# Autodesk Inventor assembly: mobile_robot_car
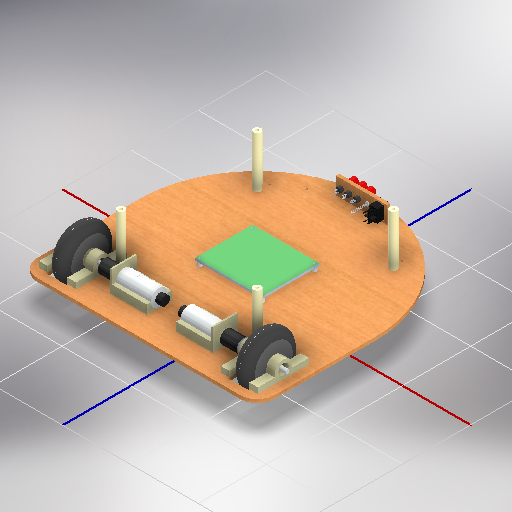
[picture p0: Inventor's stored thumbnail of the model, 512x512]
Saved by Autodesk Inventor 2026 (Build 300175050, 175E)
## iProperties
Created: 2025-06-05
Part Number: mobile_robot_car
Document SubType Name: Assembly
Designer: satom
Author: satom
## Documents named in this file (47)
- C:\Users\satom\Desktop\Robot\CAD\Inventor\mobile_robot_car.iam
- C:\Users\satom\Desktop\Robot\CAD\Inventor\C - Chassis\layer1_new.ipt
- C:\Users\satom\Desktop\Robot\CAD\Inventor\D - DriveTrain\motor_holder.ipt
- C:\Users\satom\Desktop\Robot\CAD\Inventor\D - DriveTrain\wheel_bearing.ipt
- C:\Users\satom\Desktop\Robot\CAD\Inventor\D - DriveTrain\wheel_mount.ipt
- C:\Users\satom\Desktop\Robot\CAD\Inventor\C - Chassis\3inch_standoff.ipt
- C:\Users\satom\Desktop\Robot\CAD\Inventor\solidworks\D - DriveTrain\motor\motor\motor.ipt
- C:\Users\satom\Desktop\Robot\CAD\Inventor\solidworks\D - DriveTrain\shaft_coupler\shaft_coupler\shaft_coupler.ipt
- C:\Users\satom\Desktop\Robot\CAD\Inventor\solidworks\D - DriveTrain\drive_shaft\drive_shaft\drive_shaft.ipt
- C:\Users\satom\Desktop\Robot\CAD\Inventor\solidworks\D - DriveTrain\ball_bearing\ball_bearing\ball_bearing.ipt
- C:\Users\satom\Desktop\Robot\CAD\Inventor\solidworks\E - Electronics\Main Board\Main Board\Main Board.ipt
- C:\Users\satom\Desktop\Robot\CAD\Inventor\solidworks\E - Electronics\NiMH_battery\NiMH_battery\NiMH_battery.ipt
- C:\Users\satom\Desktop\Robot\CAD\Inventor\C - Chassis\layer2_new.ipt
- C:\Users\satom\Desktop\Robot\CAD\Inventor\solidworks\E - Electronics\IMU breakout\IMU breakout\IMU breakout.ipt
- C:\Users\satom\Desktop\Robot\CAD\Inventor\C - Chassis\layer3_new.ipt
- C:\Users\satom\Desktop\Robot\CAD\Inventor\C - Chassis\9inch_spacer.ipt
- C:\Users\satom\Desktop\Robot\CAD\Inventor\C - Chassis\layer4_new.ipt
- C:\Users\satom\Desktop\Robot\CAD\Inventor\C - Chassis\layer5_new.ipt
- C:\Users\satom\Desktop\Robot\CAD\Inventor\C - Chassis\layer6_new.ipt
- C:\Users\satom\Desktop\Robot\CAD\Inventor\C - Chassis\3.5inch_standoff.ipt
- C:\Users\satom\Desktop\Robot\CAD\Inventor\solidworks\Display\Arducam_assembly\Arducam_assembly\Arducam_assembly.ipt
- C:\Users\satom\Desktop\Robot\CAD\Inventor\C - Chassis\LiDAR_plate.ipt
- C:\Users\satom\Desktop\Robot\CAD\Inventor\solidworks\E - Electronics\A2_LIDAR\A2_LIDAR\A2_LIDAR.ipt
- C:\Users\satom\Desktop\Robot\CAD\Inventor\C - Chassis\control_panel.ipt
- C:\Users\satom\Desktop\Robot\CAD\Inventor\E - Electronics\status_LED\status_LED\status_LED.ipt
- C:\Users\satom\Desktop\Robot\CAD\Inventor\E - Electronics\rocker_switch\rocker_switch\rocker_switch.ipt
- C:\Users\satom\Desktop\Robot\CAD\Inventor\E - Electronics\button\button\button.ipt
- C:\Users\satom\Desktop\Robot\CAD\Inventor\E - Electronics\microphone_casing.ipt
- C:\Users\satom\Desktop\Robot\CAD\Inventor\E - Electronics\microphone_casing_back.ipt
- C:\Users\satom\Desktop\Robot\CAD\Inventor\C - Chassis\display_top_support_left.ipt
- C:\Users\satom\Desktop\Robot\CAD\Inventor\C - Chassis\display_top_support_right.ipt
- C:\Users\satom\Desktop\Robot\CAD\Inventor\solidworks\Display\monitor\monitor\monitor.ipt
- C:\Users\satom\Desktop\Robot\CAD\Inventor\C - Chassis\display_bottom_support_left.ipt
- C:\Users\satom\Desktop\Robot\CAD\Inventor\C - Chassis\display_bottom_support_right.ipt
- C:\Users\satom\Desktop\Robot\CAD\Inventor\E - Electronics\NiMH_Holder_Front.ipt
- C:\Users\satom\Desktop\Robot\CAD\Inventor\E - Electronics\NiMH_Holder_Back.ipt
- C:\Users\satom\Desktop\Robot\CAD\Inventor\E - Electronics\jetson_orin_nano_holder_corner_1.ipt
- C:\Users\satom\Desktop\Robot\CAD\Inventor\E - Electronics\jetson_orin_nano_holder_corner_2.ipt
- C:\Users\satom\Desktop\Robot\CAD\Inventor\E - Electronics\orin_nano\orin_nano\orin_nano.ipt
- C:\Users\satom\Desktop\Robot\CAD\Inventor\E - Electronics\1-4_inch_standoff.ipt
- C:\Users\satom\Desktop\Robot\CAD\Inventor\E - Electronics\astra_holder.ipt
- C:\Users\satom\Desktop\Robot\CAD\Inventor\D - DriveTrain\wheel_80mm.ipt
- C:\Users\satom\Desktop\Robot\CAD\Inventor\D - DriveTrain\wheel_spacer_2.5mm.ipt
- C:\Users\satom\Desktop\Robot\CAD\Inventor\C - Chassis\foam_bumper_circular.ipt
- C:\Users\satom\Desktop\Robot\CAD\Inventor\C - Chassis\foam_bumper_bottom.ipt
- C:\Users\satom\Desktop\Robot\CAD\Inventor\solidworks\E - Electronics\Lion_5V\Lion_5V\Lion_5V.ipt
- C:\Users\satom\Desktop\Robot\CAD\Inventor\C - Chassis\ball_caster.ipt
## Components (103 placed, 46 different names)
1. layer1_new:1 — Mate:1, Mate:2, Mate:3, Mate:4, Mate:5, Mate:6, Mate:8, Mate:9, Mate:10, Mate:11, Mate:12, Mate:13, Mate:14, Mate:15, Mate:18, Mate:19, Mate:20, Mate:21, Mate:22, Mate:23, Mate:24, Mate:25, Mate:33, Mate:34, Mate:210, Mate:211, Mate:212, Mate:297, Mate:298, Mate:299, Mate:300, Mate:301, Mate:302, Mate:303, Mate:304, Mate:348, Mate:349, Mate:350, Mate:351, Mate:352, Mate:353
2. motor_holder:1 — Mate:1, Mate:29, Mate:30, Mate:34
3. motor_holder:2 — Mate:2, Mate:31, Mate:32, Mate:33
4. wheel_bearing:1 — Mate:5, Mate:12, Mate:13, Mate:43, Mate:44
5. wheel_bearing:2 — Mate:6, Mate:10, Mate:11, Mate:50, Mate:51
6. wheel_bearing:3 — Mate:4, Mate:14, Mate:15, Mate:45, Mate:46
7. wheel_bearing:4 — Mate:3, Mate:8, Mate:9, Mate:48, Mate:49
8. wheel_mount:1 — Mate:62, Mate:321, Mate:323
9. wheel_mount:2 — Mate:64, Mate:322, Mate:324
10. wheel_mount:3 — Mate:325, Mate:326
11. wheel_mount:4 — Mate:61, Mate:63, Mate:327, Mate:328
12. 3inch_standoff:1 — Mate:18, Mate:24, Mate:82
13. 3inch_standoff:2 — Mate:19, Mate:25, Mate:79, Mate:81
14. 3inch_standoff:3 — Mate:21, Mate:23, Mate:83
15. 3inch_standoff:4 — Mate:20, Mate:22, Mate:80
16. motor:1 — Mate:29, Mate:30, Mate:35, Mate:37
17. motor:2 — Mate:31, Mate:32, Mate:36, Mate:38
18. shaft_coupler:1 — Mate:36, Mate:38, Mate:39, Mate:41
19. shaft_coupler:2 — Mate:35, Mate:37, Mate:40, Mate:42
20. drive_shaft:1 — Mate:39, Mate:41, Mate:62, Mate:329, Mate:330
21. drive_shaft:2 — Mate:40, Mate:42, Mate:61, Mate:333, Mate:334
22. ball_bearing:1 — Mate:50, Mate:51, Mate:331
23. ball_bearing:2 — Mate:45, Mate:46, Mate:335
24. ball_bearing:3 — Mate:43, Mate:44, Mate:63, Mate:336
25. ball_bearing:4 — Mate:48, Mate:49, Mate:64, Mate:332
26. Main Board:1 — Mate:305, Mate:306, Mate:307
27. NiMH_battery:1 — Mate:265, Mate:266
28. NiMH_battery:2 — Mate:273, Mate:274
29. layer2_new:1 — Mate:79, Mate:80, Mate:81, Mate:82, Mate:83, Mate:95, Mate:96, Mate:97, Mate:98, Mate:99, Mate:100, Mate:101, Mate:102, Mate:259, Mate:260, Mate:261, Mate:262, Mate:263, Mate:264, Mate:267, Mate:268, Mate:269, Mate:270, Mate:271, Mate:272, Mate:275, Mate:276, Mate:277, Mate:282, Mate:283, Mate:284, Mate:285, Mate:286, Mate:287, Mate:288, Mate:289, Mate:290, Mate:308, Mate:309, Mate:310, Mate:311, Mate:312, Mate:313, Mate:345, Mate:346, Mate:347, Mate:354
30. IMU breakout:1 — Mate:314, Mate:315, Mate:316, Mate:317
31. 3inch_standoff:5 — Mate:97, Mate:101, Mate:103, Mate:104
32. 3inch_standoff:6 — Mate:96, Mate:102
33. 3inch_standoff:7 — Mate:98, Mate:99
34. 3inch_standoff:8 — Mate:95, Mate:100, Mate:105
35. layer3_new:1 — Mate:103, Mate:104, Mate:105, Mate:106, Mate:107, Mate:108, Mate:109, Mate:110, Mate:111, Mate:112, Mate:113, Mate:114, Mate:115, Mate:116, Mate:117, Mate:118, Mate:119, Mate:120, Mate:121, Mate:337, Mate:338
36. 9inch_spacer:1 — Mate:106, Mate:116, Mate:117, Mate:118, Mate:126, Mate:127
37. 9inch_spacer:2 — Mate:107, Mate:119, Mate:120, Mate:121, Mate:122, Mate:123, Mate:124, Mate:125
38. 9inch_spacer:3 — Mate:108, Mate:110, Mate:111, Mate:112, Mate:130, Mate:131
39. 9inch_spacer:4 — Mate:109, Mate:113, Mate:114, Mate:115, Mate:128, Mate:129
40. layer4_new:1 — Mate:122, Mate:123, Mate:124, Mate:125, Mate:126, Mate:127, Mate:128, Mate:129, Mate:130, Mate:131, Mate:132, Mate:133, Mate:134, Mate:135, Mate:136, Mate:137, Mate:138, Mate:139, Mate:140, Mate:141, Mate:142, Mate:143, Mate:144, Mate:145, Mate:146, Mate:147, Mate:339, Mate:340
41. 9inch_spacer:5 — Mate:135, Mate:145, Mate:146, Mate:147, Mate:148, Mate:152, Mate:153, Mate:154
42. 9inch_spacer:6 — Mate:134, Mate:142, Mate:143, Mate:144, Mate:155, Mate:156, Mate:157
43. 9inch_spacer:7 — Mate:133, Mate:136, Mate:137, Mate:138, Mate:158, Mate:159, Mate:160
44. 9inch_spacer:8 — Mate:132, Mate:139, Mate:140, Mate:141, Mate:149, Mate:150, Mate:151
45. layer5_new:1 — Mate:148, Mate:149, Mate:150, Mate:151, Mate:152, Mate:153, Mate:154, Mate:155, Mate:156, Mate:157, Mate:158, Mate:159, Mate:160, Mate:161, Mate:162, Mate:163, Mate:164, Mate:165, Mate:166, Mate:167, Mate:168, Mate:169, Mate:170, Mate:171, Mate:172, Mate:173, Mate:174, Mate:175, Mate:176, Mate:341, Mate:342
46. 9inch_spacer:9 — Mate:161, Mate:171, Mate:172, Mate:173, Mate:177, Mate:178, Mate:179, Mate:180, Mate:232
47. 9inch_spacer:10 — Mate:162, Mate:174, Mate:175, Mate:176, Mate:181, Mate:182, Mate:183, Mate:231
48. 9inch_spacer:11 — Mate:163, Mate:168, Mate:169, Mate:170, Mate:187, Mate:188, Mate:189
49. 9inch_spacer:12 — Mate:164, Mate:165, Mate:166, Mate:167, Mate:184, Mate:185, Mate:186
50. layer6_new:1 — Mate:177, Mate:178, Mate:179, Mate:180, Mate:181, Mate:182, Mate:183, Mate:184, Mate:185, Mate:186, Mate:187, Mate:188, Mate:189, Mate:190, Mate:191, Mate:192, Mate:193, Mate:194, Mate:195, Mate:196, Mate:197, Mate:198, Mate:199, Mate:233, Mate:234, Mate:235, Mate:236, Mate:239, Mate:243, Mate:318, Mate:319, Mate:320, Mate:343, Mate:344
51. 3.5inch_standoff:1 — Mate:191, Mate:194, Mate:201
52. 3.5inch_standoff:2 — Mate:190, Mate:197, Mate:203
53. 3.5inch_standoff:3 — Mate:192, Mate:196, Mate:200, Mate:204
54. 3.5inch_standoff:4 — Mate:193, Mate:195, Mate:202
55. Arducam_assembly:1 — Mate:198, Mate:199
56. LiDAR_plate:1 — Mate:200, Mate:201, Mate:202, Mate:203, Mate:204, Mate:205, Mate:206, Mate:207, Mate:208, Mate:209
57. A2_LIDAR:1 — Mate:205, Mate:206, Mate:207, Mate:208, Mate:209
58. control_panel:1 — Mate:210, Mate:211, Mate:212, Mate:213, Mate:214, Mate:215, Mate:216, Mate:217, Mate:218, Mate:219, Mate:220, Mate:221, Mate:222, Mate:223
59. status_LED:1 — Mate:213, Mate:214
60. rocker_switch:1 — Mate:215, Mate:216, Mate:217
61. button:1 — Mate:218, Mate:219
62. button:2 — Mate:221, Mate:222
63. button:3 — Mate:220, Mate:223
64. microphone_casing:1 — Mate:225, Mate:226, Mate:227
65. microphone_casing_back:1 — Mate:225, Mate:226, Mate:227, Mate:231
66. microphone_casing:2 — Mate:228, Mate:229, Mate:230
67. microphone_casing_back:2 — Mate:228, Mate:229, Mate:230, Mate:232
68. display_top_support_left:1 — Mate:233, Mate:234, Mate:238
69. display_top_support_right:1 — Mate:235, Mate:236, Mate:237, Mate:241
70. monitor:1 — Mate:237, Mate:238, Mate:241, Mate:242, Mate:244
71. display_bottom_support_left:1 — Mate:239, Mate:242
72. display_bottom_support_right:1 — Mate:243, Mate:244
73. NiMH_Holder_Front:1 — Mate:260, Mate:263, Mate:264, Mate:265
74. NiMH_Holder_Back:1 — Mate:259, Mate:261, Mate:262, Mate:266
75. NiMH_Holder_Back:2 — Mate:267, Mate:271, Mate:272, Mate:274
76. NiMH_Holder_Front:2 — Mate:268, Mate:269, Mate:270, Mate:273
77. jetson_orin_nano_holder_corner_1:1 — Mate:276, Mate:277, Mate:283
78. jetson_orin_nano_holder_corner_1:2 — Mate:275, Mate:282, Mate:284, Mate:292
79. jetson_orin_nano_holder_corner_2:1 — Mate:286, Mate:287, Mate:288
80. jetson_orin_nano_holder_corner_2:2 — Mate:285, Mate:289, Mate:290, Mate:291, Mate:293
81. orin_nano:1 — Mate:291, Mate:292, Mate:293
82. 1-4_inch_standoff:1 — Mate:297, Mate:302
83. 1-4_inch_standoff:2 — Mate:298, Mate:304
84. 1-4_inch_standoff:3 — Mate:299, Mate:303, Mate:306
85. 1-4_inch_standoff:4 — Mate:300, Mate:301, Mate:305, Mate:307
86. 1-4_inch_standoff:5 — Mate:308, Mate:312, Mate:317
87. 1-4_inch_standoff:6 — Mate:309, Mate:313, Mate:314, Mate:316
88. 1-4_inch_standoff:7 — Mate:310, Mate:311, Mate:315
89. astra_holder:1 — Mate:318, Mate:319, Mate:320
90. wheel_80mm:1 — Mate:321, Mate:322, Mate:323, Mate:324
91. wheel_80mm:2 — Mate:325, Mate:326, Mate:327, Mate:328
92. wheel_spacer_2.5mm:1 — Mate:330, Mate:332
93. wheel_spacer_2.5mm:2 — Mate:329, Mate:331
94. wheel_spacer_2.5mm:3 — Mate:334, Mate:336
95. wheel_spacer_2.5mm:4 — Mate:333, Mate:335
96. foam_bumper_circular:1 — Mate:337, Mate:338
97. foam_bumper_circular:2 — Mate:339, Mate:340
98. foam_bumper_circular:3 — Mate:341, Mate:342
99. foam_bumper_circular:4 — Mate:343, Mate:344
100. foam_bumper_bottom:1 — Mate:345, Mate:346, Mate:347
101. Lion_5V:1 — Mate:354
102. ball_caster:1 — Mate:349, Mate:350, Mate:351
103. ball_caster:2 — Mate:348, Mate:352, Mate:353
## Relationships (290: Mate 290)
- Mate:1: layer1_new:1 ↔ motor_holder:1
- Mate:2: layer1_new:1 ↔ motor_holder:2
- Mate:3: layer1_new:1 ↔ wheel_bearing:4
- Mate:4: layer1_new:1 ↔ wheel_bearing:3
- Mate:5: layer1_new:1 ↔ wheel_bearing:1
- Mate:6: layer1_new:1 ↔ wheel_bearing:2
- Mate:8: layer1_new:1 ↔ wheel_bearing:4
- Mate:9: layer1_new:1 ↔ wheel_bearing:4
- Mate:10: layer1_new:1 ↔ wheel_bearing:2
- Mate:11: layer1_new:1 ↔ wheel_bearing:2
- Mate:12: layer1_new:1 ↔ wheel_bearing:1
- Mate:13: layer1_new:1 ↔ wheel_bearing:1
- Mate:14: layer1_new:1 ↔ wheel_bearing:3
- Mate:15: layer1_new:1 ↔ wheel_bearing:3
- Mate:18: layer1_new:1 ↔ 3inch_standoff:1
- Mate:19: layer1_new:1 ↔ 3inch_standoff:2
- Mate:20: layer1_new:1 ↔ 3inch_standoff:4
- Mate:21: layer1_new:1 ↔ 3inch_standoff:3
- Mate:22: layer1_new:1 ↔ 3inch_standoff:4
- Mate:23: layer1_new:1 ↔ 3inch_standoff:3
- Mate:24: layer1_new:1 ↔ 3inch_standoff:1
- Mate:25: layer1_new:1 ↔ 3inch_standoff:2
- Mate:29: motor_holder:1 ↔ motor:1
- Mate:30: motor_holder:1 ↔ motor:1
- Mate:31: motor_holder:2 ↔ motor:2
- Mate:32: motor_holder:2 ↔ motor:2
- Mate:33: layer1_new:1 ↔ motor_holder:2
- Mate:34: layer1_new:1 ↔ motor_holder:1
- Mate:35: motor:1 ↔ shaft_coupler:2
- Mate:36: motor:2 ↔ shaft_coupler:1
- Mate:37 (0.508 mm): motor:1 ↔ shaft_coupler:2
- Mate:38 (0.508 mm): motor:2 ↔ shaft_coupler:1
- Mate:39: shaft_coupler:1 ↔ drive_shaft:1
- Mate:40: shaft_coupler:2 ↔ drive_shaft:2
- Mate:41: shaft_coupler:1 ↔ drive_shaft:1
- Mate:42: shaft_coupler:2 ↔ drive_shaft:2
- Mate:43: wheel_bearing:1 ↔ ball_bearing:3
- Mate:44: wheel_bearing:1 ↔ ball_bearing:3
- Mate:45: wheel_bearing:3 ↔ ball_bearing:2
- Mate:46: wheel_bearing:3 ↔ ball_bearing:2
- Mate:48: wheel_bearing:4 ↔ ball_bearing:4
- Mate:49: wheel_bearing:4 ↔ ball_bearing:4
- Mate:50: wheel_bearing:2 ↔ ball_bearing:1
- Mate:51: wheel_bearing:2 ↔ ball_bearing:1
- Mate:61: wheel_mount:4 ↔ drive_shaft:2
- Mate:62: wheel_mount:1 ↔ drive_shaft:1
- Mate:63 (2.54 mm): wheel_mount:4 ↔ ball_bearing:3
- Mate:64 (2.54 mm): wheel_mount:2 ↔ ball_bearing:4
- Mate:79: 3inch_standoff:2 ↔ layer2_new:1
- Mate:80: 3inch_standoff:4 ↔ layer2_new:1
- Mate:81: 3inch_standoff:2 ↔ layer2_new:1
- Mate:82: 3inch_standoff:1 ↔ layer2_new:1
- Mate:83: 3inch_standoff:3 ↔ layer2_new:1
- Mate:95: layer2_new:1 ↔ 3inch_standoff:8
- Mate:96: layer2_new:1 ↔ 3inch_standoff:6
- Mate:97: layer2_new:1 ↔ 3inch_standoff:5
- Mate:98: layer2_new:1 ↔ 3inch_standoff:7
- Mate:99: layer2_new:1 ↔ 3inch_standoff:7
- Mate:100: layer2_new:1 ↔ 3inch_standoff:8
- Mate:101: layer2_new:1 ↔ 3inch_standoff:5
- Mate:102: layer2_new:1 ↔ 3inch_standoff:6
- Mate:103: 3inch_standoff:5 ↔ layer3_new:1
- Mate:104: 3inch_standoff:5 ↔ layer3_new:1
- Mate:105: 3inch_standoff:8 ↔ layer3_new:1
- Mate:106: layer3_new:1 ↔ 9inch_spacer:1
- Mate:107: layer3_new:1 ↔ 9inch_spacer:2
- Mate:108: layer3_new:1 ↔ 9inch_spacer:3
- Mate:109: layer3_new:1 ↔ 9inch_spacer:4
- Mate:110: layer3_new:1 ↔ 9inch_spacer:3
- Mate:111: layer3_new:1 ↔ 9inch_spacer:3
- Mate:112: layer3_new:1 ↔ 9inch_spacer:3
- Mate:113: layer3_new:1 ↔ 9inch_spacer:4
- Mate:114: layer3_new:1 ↔ 9inch_spacer:4
- Mate:115: layer3_new:1 ↔ 9inch_spacer:4
- Mate:116: layer3_new:1 ↔ 9inch_spacer:1
- Mate:117: layer3_new:1 ↔ 9inch_spacer:1
- Mate:118: layer3_new:1 ↔ 9inch_spacer:1
- Mate:119: layer3_new:1 ↔ 9inch_spacer:2
- Mate:120: layer3_new:1 ↔ 9inch_spacer:2
- Mate:121: layer3_new:1 ↔ 9inch_spacer:2
- Mate:122: 9inch_spacer:2 ↔ layer4_new:1
- Mate:123: 9inch_spacer:2 ↔ layer4_new:1
- Mate:124: 9inch_spacer:2 ↔ layer4_new:1
- Mate:125: 9inch_spacer:2 ↔ layer4_new:1
- Mate:126: 9inch_spacer:1 ↔ layer4_new:1
- Mate:127: 9inch_spacer:1 ↔ layer4_new:1
- Mate:128: 9inch_spacer:4 ↔ layer4_new:1
- Mate:129: 9inch_spacer:4 ↔ layer4_new:1
- Mate:130: 9inch_spacer:3 ↔ layer4_new:1
- Mate:131: 9inch_spacer:3 ↔ layer4_new:1
- Mate:132: layer4_new:1 ↔ 9inch_spacer:8
- Mate:133: layer4_new:1 ↔ 9inch_spacer:7
- Mate:134: layer4_new:1 ↔ 9inch_spacer:6
- Mate:135: layer4_new:1 ↔ 9inch_spacer:5
- Mate:136: layer4_new:1 ↔ 9inch_spacer:7
- Mate:137: layer4_new:1 ↔ 9inch_spacer:7
- Mate:138: layer4_new:1 ↔ 9inch_spacer:7
- Mate:139: layer4_new:1 ↔ 9inch_spacer:8
- Mate:140: layer4_new:1 ↔ 9inch_spacer:8
- Mate:141: layer4_new:1 ↔ 9inch_spacer:8
- Mate:142: layer4_new:1 ↔ 9inch_spacer:6
- Mate:143: layer4_new:1 ↔ 9inch_spacer:6
- Mate:144: layer4_new:1 ↔ 9inch_spacer:6
- Mate:145: layer4_new:1 ↔ 9inch_spacer:5
- Mate:146: layer4_new:1 ↔ 9inch_spacer:5
- Mate:147: layer4_new:1 ↔ 9inch_spacer:5
- Mate:148: 9inch_spacer:5 ↔ layer5_new:1
- Mate:149: 9inch_spacer:8 ↔ layer5_new:1
- Mate:150: 9inch_spacer:8 ↔ layer5_new:1
- Mate:151: 9inch_spacer:8 ↔ layer5_new:1
- Mate:152: 9inch_spacer:5 ↔ layer5_new:1
- Mate:153: 9inch_spacer:5 ↔ layer5_new:1
- Mate:154: 9inch_spacer:5 ↔ layer5_new:1
- Mate:155: 9inch_spacer:6 ↔ layer5_new:1
- Mate:156: 9inch_spacer:6 ↔ layer5_new:1
- Mate:157: 9inch_spacer:6 ↔ layer5_new:1
- Mate:158: 9inch_spacer:7 ↔ layer5_new:1
- Mate:159: 9inch_spacer:7 ↔ layer5_new:1
- Mate:160: 9inch_spacer:7 ↔ layer5_new:1
- Mate:161: layer5_new:1 ↔ 9inch_spacer:9
- Mate:162: layer5_new:1 ↔ 9inch_spacer:10
- Mate:163: layer5_new:1 ↔ 9inch_spacer:11
- Mate:164: layer5_new:1 ↔ 9inch_spacer:12
- Mate:165: layer5_new:1 ↔ 9inch_spacer:12
- Mate:166: layer5_new:1 ↔ 9inch_spacer:12
- Mate:167: layer5_new:1 ↔ 9inch_spacer:12
- Mate:168: layer5_new:1 ↔ 9inch_spacer:11
- Mate:169: layer5_new:1 ↔ 9inch_spacer:11
- Mate:170: layer5_new:1 ↔ 9inch_spacer:11
- Mate:171: layer5_new:1 ↔ 9inch_spacer:9
- Mate:172: layer5_new:1 ↔ 9inch_spacer:9
- Mate:173: layer5_new:1 ↔ 9inch_spacer:9
- Mate:174: layer5_new:1 ↔ 9inch_spacer:10
- Mate:175: layer5_new:1 ↔ 9inch_spacer:10
- Mate:176: layer5_new:1 ↔ 9inch_spacer:10
- Mate:177: 9inch_spacer:9 ↔ layer6_new:1
- Mate:178: 9inch_spacer:9 ↔ layer6_new:1
- Mate:179: 9inch_spacer:9 ↔ layer6_new:1
- Mate:180: 9inch_spacer:9 ↔ layer6_new:1
- Mate:181: 9inch_spacer:10 ↔ layer6_new:1
- Mate:182: 9inch_spacer:10 ↔ layer6_new:1
- Mate:183: 9inch_spacer:10 ↔ layer6_new:1
- Mate:184: 9inch_spacer:12 ↔ layer6_new:1
- Mate:185: 9inch_spacer:12 ↔ layer6_new:1
- Mate:186: 9inch_spacer:12 ↔ layer6_new:1
- Mate:187: 9inch_spacer:11 ↔ layer6_new:1
- Mate:188: 9inch_spacer:11 ↔ layer6_new:1
- Mate:189: 9inch_spacer:11 ↔ layer6_new:1
- Mate:190: layer6_new:1 ↔ 3.5inch_standoff:2
- Mate:191: layer6_new:1 ↔ 3.5inch_standoff:1
- Mate:192: layer6_new:1 ↔ 3.5inch_standoff:3
- Mate:193: layer6_new:1 ↔ 3.5inch_standoff:4
- Mate:194: layer6_new:1 ↔ 3.5inch_standoff:1
- Mate:195: layer6_new:1 ↔ 3.5inch_standoff:4
- Mate:196: layer6_new:1 ↔ 3.5inch_standoff:3
- Mate:197: layer6_new:1 ↔ 3.5inch_standoff:2
- Mate:198: layer6_new:1 ↔ Arducam_assembly:1
- Mate:199: layer6_new:1 ↔ Arducam_assembly:1
- Mate:200: 3.5inch_standoff:3 ↔ LiDAR_plate:1
- Mate:201: 3.5inch_standoff:1 ↔ LiDAR_plate:1
- Mate:202: 3.5inch_standoff:4 ↔ LiDAR_plate:1
- Mate:203: 3.5inch_standoff:2 ↔ LiDAR_plate:1
- Mate:204: 3.5inch_standoff:3 ↔ LiDAR_plate:1
- Mate:205: LiDAR_plate:1 ↔ A2_LIDAR:1
- Mate:206: LiDAR_plate:1 ↔ A2_LIDAR:1
- Mate:207: LiDAR_plate:1 ↔ A2_LIDAR:1
- Mate:208: LiDAR_plate:1 ↔ A2_LIDAR:1
- Mate:209: LiDAR_plate:1 ↔ A2_LIDAR:1
- Mate:210: layer1_new:1 ↔ control_panel:1
- Mate:211: layer1_new:1 ↔ control_panel:1
- Mate:212: layer1_new:1 ↔ control_panel:1
- Mate:213: control_panel:1 ↔ status_LED:1
- Mate:214: control_panel:1 ↔ status_LED:1
- Mate:215: control_panel:1 ↔ rocker_switch:1
- Mate:216: control_panel:1 ↔ rocker_switch:1
- Mate:217: control_panel:1 ↔ rocker_switch:1
- Mate:218: control_panel:1 ↔ button:1
- Mate:219: control_panel:1 ↔ button:1
- Mate:220: control_panel:1 ↔ button:3
- Mate:221: control_panel:1 ↔ button:2
- Mate:222: control_panel:1 ↔ button:2
- Mate:223: control_panel:1 ↔ button:3
- Mate:225: microphone_casing:1 ↔ microphone_casing_back:1
- Mate:226: microphone_casing:1 ↔ microphone_casing_back:1
- Mate:227: microphone_casing:1 ↔ microphone_casing_back:1
- Mate:228: microphone_casing:2 ↔ microphone_casing_back:2
- Mate:229: microphone_casing:2 ↔ microphone_casing_back:2
- Mate:230: microphone_casing:2 ↔ microphone_casing_back:2
- Mate:231: 9inch_spacer:10 ↔ microphone_casing_back:1
- Mate:232: 9inch_spacer:9 ↔ microphone_casing_back:2
- Mate:233: layer6_new:1 ↔ display_top_support_left:1
- Mate:234: layer6_new:1 ↔ display_top_support_left:1
- Mate:235: layer6_new:1 ↔ display_top_support_right:1
- Mate:236: layer6_new:1 ↔ display_top_support_right:1
- Mate:237: display_top_support_right:1 ↔ monitor:1
- Mate:238: display_top_support_left:1 ↔ monitor:1
- Mate:239: layer6_new:1 ↔ display_bottom_support_left:1
- Mate:241: display_top_support_right:1 ↔ monitor:1
- Mate:242: monitor:1 ↔ display_bottom_support_left:1
- Mate:243: layer6_new:1 ↔ display_bottom_support_right:1
- Mate:244: monitor:1 ↔ display_bottom_support_right:1
- Mate:259: layer2_new:1 ↔ NiMH_Holder_Back:1
- Mate:260: layer2_new:1 ↔ NiMH_Holder_Front:1
- Mate:261: layer2_new:1 ↔ NiMH_Holder_Back:1
- Mate:262: layer2_new:1 ↔ NiMH_Holder_Back:1
- Mate:263: layer2_new:1 ↔ NiMH_Holder_Front:1
- Mate:264: layer2_new:1 ↔ NiMH_Holder_Front:1
- Mate:265: NiMH_battery:1 ↔ NiMH_Holder_Front:1
- Mate:266: NiMH_battery:1 ↔ NiMH_Holder_Back:1
- Mate:267: layer2_new:1 ↔ NiMH_Holder_Back:2
- Mate:268: layer2_new:1 ↔ NiMH_Holder_Front:2
- Mate:269: layer2_new:1 ↔ NiMH_Holder_Front:2
- Mate:270: layer2_new:1 ↔ NiMH_Holder_Front:2
- Mate:271: layer2_new:1 ↔ NiMH_Holder_Back:2
- Mate:272: layer2_new:1 ↔ NiMH_Holder_Back:2
- Mate:273: NiMH_battery:2 ↔ NiMH_Holder_Front:2
- Mate:274: NiMH_battery:2 ↔ NiMH_Holder_Back:2
- Mate:275: layer2_new:1 ↔ jetson_orin_nano_holder_corner_1:2
- Mate:276: layer2_new:1 ↔ jetson_orin_nano_holder_corner_1:1
- Mate:277: layer2_new:1 ↔ jetson_orin_nano_holder_corner_1:1
- Mate:282: layer2_new:1 ↔ jetson_orin_nano_holder_corner_1:2
- Mate:283: layer2_new:1 ↔ jetson_orin_nano_holder_corner_1:1
- Mate:284: layer2_new:1 ↔ jetson_orin_nano_holder_corner_1:2
- Mate:285: layer2_new:1 ↔ jetson_orin_nano_holder_corner_2:2
- Mate:286: layer2_new:1 ↔ jetson_orin_nano_holder_corner_2:1
- Mate:287: layer2_new:1 ↔ jetson_orin_nano_holder_corner_2:1
- Mate:288: layer2_new:1 ↔ jetson_orin_nano_holder_corner_2:1
- Mate:289: layer2_new:1 ↔ jetson_orin_nano_holder_corner_2:2
- Mate:290: layer2_new:1 ↔ jetson_orin_nano_holder_corner_2:2
- Mate:291: jetson_orin_nano_holder_corner_2:2 ↔ orin_nano:1
- Mate:292: jetson_orin_nano_holder_corner_1:2 ↔ orin_nano:1
- Mate:293: jetson_orin_nano_holder_corner_2:2 ↔ orin_nano:1
- Mate:297: layer1_new:1 ↔ 1-4_inch_standoff:1
- Mate:298: layer1_new:1 ↔ 1-4_inch_standoff:2
- Mate:299: layer1_new:1 ↔ 1-4_inch_standoff:3
- Mate:300: layer1_new:1 ↔ 1-4_inch_standoff:4
- Mate:301: layer1_new:1 ↔ 1-4_inch_standoff:4
- Mate:302: layer1_new:1 ↔ 1-4_inch_standoff:1
- Mate:303: layer1_new:1 ↔ 1-4_inch_standoff:3
- Mate:304: layer1_new:1 ↔ 1-4_inch_standoff:2
- Mate:305: Main Board:1 ↔ 1-4_inch_standoff:4
- Mate:306: Main Board:1 ↔ 1-4_inch_standoff:3
- Mate:307: Main Board:1 ↔ 1-4_inch_standoff:4
- Mate:308: layer2_new:1 ↔ 1-4_inch_standoff:5
- Mate:309: layer2_new:1 ↔ 1-4_inch_standoff:6
- Mate:310: layer2_new:1 ↔ 1-4_inch_standoff:7
- Mate:311: layer2_new:1 ↔ 1-4_inch_standoff:7
- Mate:312: layer2_new:1 ↔ 1-4_inch_standoff:5
- Mate:313: layer2_new:1 ↔ 1-4_inch_standoff:6
- Mate:314: IMU breakout:1 ↔ 1-4_inch_standoff:6
- Mate:315: IMU breakout:1 ↔ 1-4_inch_standoff:7
- Mate:316: IMU breakout:1 ↔ 1-4_inch_standoff:6
- Mate:317: IMU breakout:1 ↔ 1-4_inch_standoff:5
- Mate:318: layer6_new:1 ↔ astra_holder:1
- Mate:319: layer6_new:1 ↔ astra_holder:1
- Mate:320: layer6_new:1 ↔ astra_holder:1
- Mate:321: wheel_mount:1 ↔ wheel_80mm:1
- Mate:322: wheel_mount:2 ↔ wheel_80mm:1
- Mate:323: wheel_mount:1 ↔ wheel_80mm:1
- Mate:324: wheel_mount:2 ↔ wheel_80mm:1
- Mate:325: wheel_mount:3 ↔ wheel_80mm:2
- Mate:326: wheel_mount:3 ↔ wheel_80mm:2
- Mate:327: wheel_mount:4 ↔ wheel_80mm:2
- Mate:328: wheel_mount:4 ↔ wheel_80mm:2
- Mate:329: drive_shaft:1 ↔ wheel_spacer_2.5mm:2
- Mate:330: drive_shaft:1 ↔ wheel_spacer_2.5mm:1
- Mate:331: ball_bearing:1 ↔ wheel_spacer_2.5mm:2
- Mate:332: ball_bearing:4 ↔ wheel_spacer_2.5mm:1
- Mate:333: drive_shaft:2 ↔ wheel_spacer_2.5mm:4
- Mate:334: drive_shaft:2 ↔ wheel_spacer_2.5mm:3
- Mate:335: ball_bearing:2 ↔ wheel_spacer_2.5mm:4
- Mate:336: ball_bearing:3 ↔ wheel_spacer_2.5mm:3
- Mate:337: layer3_new:1 ↔ foam_bumper_circular:1
- Mate:338: layer3_new:1 ↔ foam_bumper_circular:1
- Mate:339: layer4_new:1 ↔ foam_bumper_circular:2
- Mate:340: layer4_new:1 ↔ foam_bumper_circular:2
- Mate:341: layer5_new:1 ↔ foam_bumper_circular:3
- Mate:342: layer5_new:1 ↔ foam_bumper_circular:3
- Mate:343: layer6_new:1 ↔ foam_bumper_circular:4
- Mate:344: layer6_new:1 ↔ foam_bumper_circular:4
- Mate:345: layer2_new:1 ↔ foam_bumper_bottom:1
- Mate:346: layer2_new:1 ↔ foam_bumper_bottom:1
- Mate:347: layer2_new:1 ↔ foam_bumper_bottom:1
- Mate:348: layer1_new:1 ↔ ball_caster:2
- Mate:349: layer1_new:1 ↔ ball_caster:1
- Mate:350: layer1_new:1 ↔ ball_caster:1
- Mate:351: layer1_new:1 ↔ ball_caster:1
- Mate:352: layer1_new:1 ↔ ball_caster:2
- Mate:353: layer1_new:1 ↔ ball_caster:2
- Mate:354: layer2_new:1 ↔ Lion_5V:1
## Named parameters: m3_heat_set_insert = 4 mm
